# Autodesk Inventor assembly: assembly
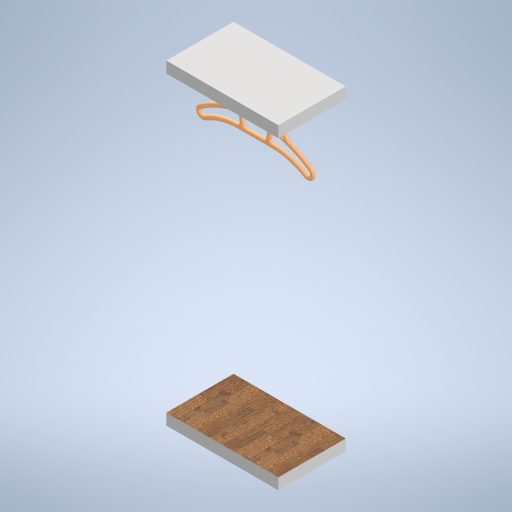
[picture p0: Inventor's stored thumbnail of the model, 512x512]
Saved by Autodesk Inventor 2024 (Build 280153020, 153B)
## iProperties
Created: 2023-05-23
Part Number: assembly
Document SubType Name: Assembly
Designer: Patrick
Author: Patrick
## Documents named in this file (8)
- C:\Users\Patrick\source\Private\pull-up-bar\cad\main.iam
- C:\Users\Patrick\source\Private\pull-up-bar\cad\ring.iam
- C:\Users\Patrick\source\Private\pull-up-bar\cad\bar.ipt
- C:\Users\Patrick\source\Private\pull-up-bar\cad\hook.ipt
- C:\Users\Patrick\source\Private\pull-up-bar\cad\ground.ipt
- C:\Users\Patrick\source\Private\pull-up-bar\cad\ceiling.ipt
- C:\Users\Patrick\source\Private\pull-up-bar\cad\carabiner.ipt
- C:\Users\Patrick\source\Private\pull-up-bar\cad\ISO 4017 - M8 x 50 - ISO.ipt
## Components (13 placed, 7 different names)
1. ceiling:1 — Mate:20, Mate:28
2. hook:1 — Mate:14, Insert:1, Insert:2
3. hook:2 — Mate:27, Mate:28, Mate:29, Insert:3, Insert:4
4. ISO 4017 M8 x 50:5 — Insert:1
5. ISO 4017 M8 x 50:6 — Insert:2
6. ISO 4017 M8 x 50:7 — Insert:3
7. ISO 4017 M8 x 50:8 — Insert:4
8. carabiner:1
9. carabiner:2
10. bar:1 — Flush:11, Mate:29, Flush:25
11. ring:1 [sub-assembly] — Angle:1, Flush:12, Flush:13
12. ring:2 [sub-assembly] — Flush:24, Mate:27
13. ground:1 — Flush:17, Flush:19, Flush:20, Mate:20
## Relationships (33: Mate 15, Flush 13, Insert 4, Angle 1)
- [Flush]: bar:1
- [Mate]: carabiner:1
- Angle:1 (0 deg): ring:1
- Flush:11: bar:1
- Flush:12 (-250 mm): ring:1
- Flush:13: ring:1
- Mate:14: hook:1
- [Mate] (5 mm): hook:1 ↔ carabiner:1
- [Mate]: hook:1 ↔ carabiner:1
- [Mate]: ceiling:1 ↔ hook:1
- Flush:17: ground:1
- [Flush]: ceiling:1
- Flush:19: ground:1
- Flush:20: ground:1
- [Flush]: ceiling:1
- Mate:20 (2620 mm): ceiling:1 ↔ ground:1
- [Flush]: carabiner:1 ↔ ring:1
- [Mate]: carabiner:1 ↔ ring:1
- [Mate]: carabiner:1 ↔ ring:1
- [Mate] (5 mm): hook:2 ↔ carabiner:2
- [Mate]: hook:2 ↔ carabiner:2
- [Flush]: carabiner:2 ↔ ring:2
- [Mate]: carabiner:2 ↔ ring:2
- [Mate]: carabiner:2 ↔ ring:2
- Flush:24: ring:2
- Mate:27: hook:2 ↔ ring:2
- Mate:28: ceiling:1 ↔ hook:2
- Mate:29: hook:2 ↔ bar:1
- Insert:1: hook:1 ↔ ISO 4017 M8 x 50:5
- Insert:2: hook:1 ↔ ISO 4017 M8 x 50:6
- Insert:3: hook:2 ↔ ISO 4017 M8 x 50:7
- Insert:4: hook:2 ↔ ISO 4017 M8 x 50:8
- Flush:25 (-2260 mm): bar:1
## Named parameters: d77_d62 = 5 mm, d78_d63 = 0 mm, d79_d31 = 0 mm, d80_d32 = 0 mm, d81_d7 = 0 mm
